# Autodesk Inventor assembly: camera_module
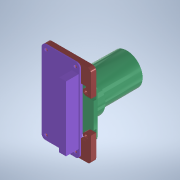
[picture p0: Inventor's stored thumbnail of the model, 180x180]
Saved by Autodesk Inventor 2021 (Build 250183000, 183)
## iProperties
Created: 2021-02-15
Part Number: camera_module
Document SubType Name: Assembly
Designer: lobato
Author: lobato
## Documents named in this file (4)
- C:\Users\lobato\Desktop\LiftPose3d-device\v2_raspberry\camera_module.iam
- C:\Users\lobato\Desktop\LiftPose3d-device\v2_raspberry\coupler.ipt
- C:\Users\lobato\Desktop\LiftPose3d-device\v2_raspberry\camera.ipt
- C:\Users\lobato\Desktop\LiftPose3d-device\v2_raspberry\raspberry.ipt
## Components (3 placed, 3 different names)
1. coupler:1 — Insert:1, Insert:2, Insert:3, Insert:4
2. camera:1 — Insert:1, Insert:2
3. raspberry:1 — Insert:3, Insert:4
## Relationships (4: Insert 4)
- Insert:1: coupler:1 ↔ camera:1
- Insert:2: coupler:1 ↔ camera:1
- Insert:3: coupler:1 ↔ raspberry:1
- Insert:4: coupler:1 ↔ raspberry:1
